# Autodesk Inventor assembly: eje
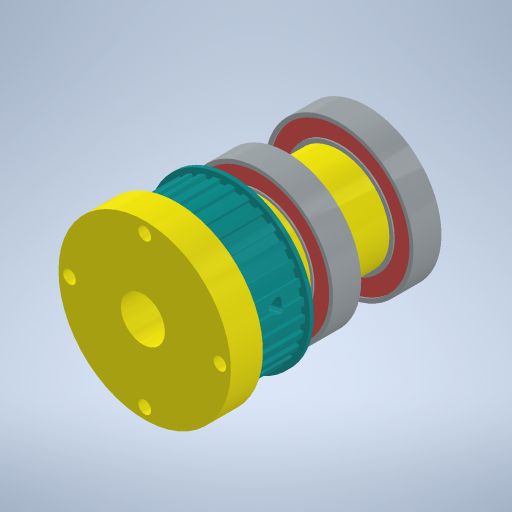
[picture p0: Inventor's stored thumbnail of the model, 512x512]
Saved by Autodesk Inventor 2024.3 (Build 283343000, 343)
## iProperties
Created: 2024-09-30
Part Number: eje
Document SubType Name: Assembly
Designer: User
Author: User
## Documents named in this file (4)
- C:\Users\User\Documents\Universidad Octavo Semestre\Robotica Industrial\matlab\SCARA\mariana_scara_final\mariana_scara_final\eje.iam
- C:\Users\User\Documents\Universidad Octavo Semestre\Robotica Industrial\matlab\SCARA\mariana_scara_final\mariana_scara_final\eje_25.ipt
- C:\Users\User\Documents\Universidad Octavo Semestre\Robotica Industrial\matlab\SCARA\mariana_scara_final\mariana_scara_final\polea.ipt
- C:\Users\User\Documents\Universidad Octavo Semestre\Robotica Industrial\matlab\SCARA\mariana_scara_final\mariana_scara_final\rodamiento-25-37-7.ipt
## Components (4 placed, 3 different names)
1. eje_25:1 — Insert:1, Insert:2, Insert:3
2. polea:1 — Insert:1
3. rodamiento-25-37-7:1 — Insert:2
4. rodamiento-25-37-7:2 — Insert:3
## Relationships (3: Insert 3)
- Insert:1: eje_25:1 ↔ polea:1
- Insert:2: eje_25:1 ↔ rodamiento-25-37-7:1
- Insert:3: eje_25:1 ↔ rodamiento-25-37-7:2
